# Autodesk Inventor assembly: BoronProbe_5_disassembled
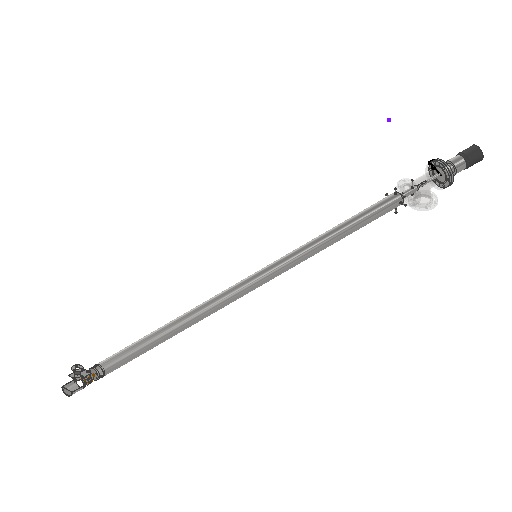
[picture p0: Inventor's stored thumbnail of the model, 512x512]
Saved by Autodesk Inventor 2026.2 (Build 302298000, 298)
## iProperties
Created: 2026-05-08
Part Number: BoronProbe_5_disassembled
Document SubType Name: Assembly
Designer: zetsu
Author: zetsu
## Documents named in this file (20)
- D:\repos\PIHTI\BoronProbe_5\BoronProbe_5_disassembled.iam
- D:\repos\PIHTI\BoronProbe_5\parts\B_probehead_5.ipt
- D:\repos\PIHTI\BoronProbe_5\parts\B_holder_sub_5.ipt
- D:\repos\PIHTI\BoronProbe_5\parts\B_pipe_cylinder_5.ipt
- D:\repos\PIHTI\BoronProbe_5\parts\B_holder_up_5.ipt
- D:\repos\PIHTI\BoronProbe_5\parts\M3-nut.ipt
- D:\repos\PIHTI\BoronProbe_5\parts\M3x6-BHCS.ipt
- D:\repos\PIHTI\BoronProbe_5\parts\substrate.ipt
- D:\repos\PIHTI\BoronProbe_5\parts\ceramic_bushing_M3-v1.ipt
- D:\repos\PIHTI\BoronProbe_5\parts\ceramic_washer_M4_v1.ipt
- D:\repos\PIHTI\BoronProbe_5\parts\B_probe_pipe_5.ipt
- D:\repos\PIHTI\BoronProbe_5\parts\B_shield_5.iam
- D:\repos\PIHTI\BoronProbe_5\parts\ceramic_2-hole-spacer_d3-13.ipt
- D:\repos\PIHTI\BoronProbe_5\parts\ceramic_spacer_d3-13.ipt
- D:\repos\PIHTI\BoronProbe_5\parts\M2-4_screw.ipt
- D:\repos\PIHTI\BoronProbe_5\parts\rotary_transfer_shaft_5.ipt
- D:\repos\PIHTI\BoronProbe_5\parts\M3x10-BHCS.ipt
- D:\repos\PIHTI\BoronProbe_5\parts\Rotary_Feedthrough\Rotary_Feedthrough.iam
- D:\repos\PIHTI\BoronProbe_5\parts\M3x20-BHCS.ipt
- D:\repos\PIHTI\BoronProbe_5\parts\ICF70TE\ICF70TE.iam
## Components (38 placed, 17 different names)
1. B_probehead_5:1 — メイト:1, メイト:2, メイト:3, メイト:4, メイト:6, メイト:12, メイト:13, メイト:14, メイト:15, メイト:16, メイト:17, メイト:18, メイト:20, メイト:22, メイト:49, メイト:50, メイト:51, メイト:52, フラッシュ:1, メイト:53, フラッシュ:2, メイト:54, フラッシュ:3
2. B_holder_sub_5:1 — メイト:1, メイト:2, メイト:3, メイト:5, メイト:7, メイト:63, メイト:64, メイト:65, メイト:66, メイト:67, メイト:68, メイト:69, メイト:70
3. Broached Hexagon Socket Button Head Cap Screw - Metric M3 x 0.5 x 6:1 — メイト:4, メイト:5
4. Broached Hexagon Socket Button Head Cap Screw - Metric M3 x 0.5 x 6:2 — メイト:6, メイト:7
5. Broached Hexagon Socket Button Head Cap Screw - Metric M3 x 0.5 x 6:5 — メイト:40, メイト:41
6. ceramic_bushing_M3-v1:1 — メイト:16, メイト:17, メイト:23, メイト:36, メイト:37
7. ceramic_bushing_M3-v1:2 — メイト:14, メイト:15, メイト:19, メイト:40, メイト:41
8. ceramic_bushing_M3-v1:3 — メイト:12, メイト:13, メイト:21, メイト:38, メイト:39
9. ceramic_washer_M4_v1:1 — メイト:20, メイト:21, メイト:43
10. ceramic_washer_M4_v1:2 — メイト:18, メイト:19, メイト:42
11. ceramic_washer_M4_v1:3 — メイト:22, メイト:23, メイト:44
12. Broached Hexagon Socket Button Head Cap Screw - Metric M3 x 0.5 x 6:6 — メイト:38, メイト:39
13. Broached Hexagon Socket Button Head Cap Screw - Metric M3 x 0.5 x 6:7 — メイト:36, メイト:37
14. B_probe_pipe_5:1 — メイト:45, メイト:46, メイト:79, メイト:80, メイト:81, メイト:82, メイト:83
15. B_pipe_cylinder_5:1 — メイト:42, メイト:43, メイト:44, メイト:45, メイト:46
16. B_shield_5:1 [sub-assembly] — メイト:49, メイト:50, メイト:51, メイト:55, メイト:56, メイト:77, メイト:78
17. ceramic_2-hole-spacer_d3-13:1 — メイト:54, フラッシュ:3
18. ceramic_spacer_d3-13:1 — メイト:53, フラッシュ:2
19. ceramic_spacer_d3-13:2 — メイト:52, フラッシュ:1
20. M2-4_screw:1 — メイト:55, メイト:77
21. M2-4_screw:2 — メイト:56, メイト:78
22. JIS B 1181 Style 1 - Metric A M3:1 — メイト:63, メイト:64
23. JIS B 1181 Style 1 - Metric A M3:2 — メイト:65, メイト:66
24. JIS B 1181 Style 1 - Metric A M3:3 — メイト:67, メイト:68
25. substrate:1 — メイト:69
26. B_holder_up_5:1 — メイト:70, メイト:71, メイト:72, メイト:73, メイト:74, メイト:75, メイト:76
27. Broached Hexagon Socket Button Head Cap Screw - Metric M3 x 0.5 x 6:8 — メイト:71, メイト:72
28. Broached Hexagon Socket Button Head Cap Screw - Metric M3 x 0.5 x 6:9 — メイト:73, メイト:74
29. Broached Hexagon Socket Button Head Cap Screw - Metric M3 x 0.5 x 6:10 — メイト:75, メイト:76
30. rotary_transfer_shaft_5:1 — メイト:79, メイト:84, 角度:1, メイト:85
31. Broached Hexagon Socket Button Head Cap Screw - Metric M3 x 0.5 x 6:11 — メイト:80
32. Broached Hexagon Socket Button Head Cap Screw - Metric M3 x 0.5 x 6:12 — メイト:81
33. Broached Hexagon Socket Button Head Cap Screw - Metric M3 x 0.5 x 6:13 — メイト:82
34. Broached Hexagon Socket Button Head Cap Screw - Metric M3 x 0.5 x 6:14 — メイト:83
35. Rotary_Feedthrough:1 [sub-assembly] — メイト:84, 角度:1, メイト:87, メイト:88, メイト:89
36. Broached Hexagon Socket Button Head Cap Screw - Metric M3 x 0.5 x 6:15 — メイト:85, メイト:86
37. JIS B 1181 Style 1 - Metric A M3:4 — メイト:86
38. ICF70TE:1 [sub-assembly] — メイト:87, メイト:88, メイト:89
## Relationships (69: Mate 65, Flush 3, Angle 1)
- メイト:1 [Mate]: B_probehead_5:1 ↔ B_holder_sub_5:1
- メイト:2 [Mate]: B_probehead_5:1 ↔ B_holder_sub_5:1
- メイト:3 [Mate]: B_probehead_5:1 ↔ B_holder_sub_5:1
- メイト:4 [Mate]: B_probehead_5:1 ↔ Broached Hexagon Socket Button Head Cap Screw - Metric M3 x 0.5 x 6:1
- メイト:5 [Mate]: B_holder_sub_5:1 ↔ Broached Hexagon Socket Button Head Cap Screw - Metric M3 x 0.5 x 6:1
- メイト:6 [Mate]: B_probehead_5:1 ↔ Broached Hexagon Socket Button Head Cap Screw - Metric M3 x 0.5 x 6:2
- メイト:7 [Mate]: B_holder_sub_5:1 ↔ Broached Hexagon Socket Button Head Cap Screw - Metric M3 x 0.5 x 6:2
- メイト:12 [Mate]: B_probehead_5:1 ↔ ceramic_bushing_M3-v1:3
- メイト:13 [Mate]: B_probehead_5:1 ↔ ceramic_bushing_M3-v1:3
- メイト:14 [Mate]: B_probehead_5:1 ↔ ceramic_bushing_M3-v1:2
- メイト:15 [Mate]: B_probehead_5:1 ↔ ceramic_bushing_M3-v1:2
- メイト:16 [Mate]: B_probehead_5:1 ↔ ceramic_bushing_M3-v1:1
- メイト:17 [Mate]: B_probehead_5:1 ↔ ceramic_bushing_M3-v1:1
- メイト:18 [Mate]: B_probehead_5:1 ↔ ceramic_washer_M4_v1:2
- メイト:19 [Mate]: ceramic_bushing_M3-v1:2 ↔ ceramic_washer_M4_v1:2
- メイト:20 [Mate]: B_probehead_5:1 ↔ ceramic_washer_M4_v1:1
- メイト:21 [Mate]: ceramic_bushing_M3-v1:3 ↔ ceramic_washer_M4_v1:1
- メイト:22 [Mate]: B_probehead_5:1 ↔ ceramic_washer_M4_v1:3
- メイト:23 [Mate]: ceramic_bushing_M3-v1:1 ↔ ceramic_washer_M4_v1:3
- メイト:36 [Mate]: ceramic_bushing_M3-v1:1 ↔ Broached Hexagon Socket Button Head Cap Screw - Metric M3 x 0.5 x 6:7
- メイト:37 [Mate]: ceramic_bushing_M3-v1:1 ↔ Broached Hexagon Socket Button Head Cap Screw - Metric M3 x 0.5 x 6:7
- メイト:38 [Mate]: ceramic_bushing_M3-v1:3 ↔ Broached Hexagon Socket Button Head Cap Screw - Metric M3 x 0.5 x 6:6
- メイト:39 [Mate]: ceramic_bushing_M3-v1:3 ↔ Broached Hexagon Socket Button Head Cap Screw - Metric M3 x 0.5 x 6:6
- メイト:40 [Mate]: Broached Hexagon Socket Button Head Cap Screw - Metric M3 x 0.5 x 6:5 ↔ ceramic_bushing_M3-v1:2
- メイト:41 [Mate]: Broached Hexagon Socket Button Head Cap Screw - Metric M3 x 0.5 x 6:5 ↔ ceramic_bushing_M3-v1:2
- メイト:42 [Mate]: ceramic_washer_M4_v1:2 ↔ B_pipe_cylinder_5:1
- メイト:43 [Mate]: ceramic_washer_M4_v1:1 ↔ B_pipe_cylinder_5:1
- メイト:44 [Mate]: ceramic_washer_M4_v1:3 ↔ B_pipe_cylinder_5:1
- メイト:45 [Mate]: B_probe_pipe_5:1 ↔ B_pipe_cylinder_5:1
- メイト:46 [Mate]: B_probe_pipe_5:1 ↔ B_pipe_cylinder_5:1
- メイト:49 [Mate]: B_probehead_5:1 ↔ B_shield_5:1
- メイト:50 [Mate]: B_probehead_5:1 ↔ B_shield_5:1
- メイト:51 [Mate]: B_probehead_5:1 ↔ B_shield_5:1
- メイト:52 [Mate]: B_probehead_5:1 ↔ ceramic_spacer_d3-13:2
- フラッシュ:1 [Flush]: B_probehead_5:1 ↔ ceramic_spacer_d3-13:2
- メイト:53 [Mate]: B_probehead_5:1 ↔ ceramic_spacer_d3-13:1
- フラッシュ:2 [Flush]: B_probehead_5:1 ↔ ceramic_spacer_d3-13:1
- メイト:54 [Mate]: B_probehead_5:1 ↔ ceramic_2-hole-spacer_d3-13:1
- フラッシュ:3 [Flush]: B_probehead_5:1 ↔ ceramic_2-hole-spacer_d3-13:1
- メイト:55 [Mate]: B_shield_5:1 ↔ M2-4_screw:1
- メイト:56 [Mate]: B_shield_5:1 ↔ M2-4_screw:2
- メイト:63 [Mate]: B_holder_sub_5:1 ↔ JIS B 1181 Style 1 - Metric A M3:1
- メイト:64 [Mate]: B_holder_sub_5:1 ↔ JIS B 1181 Style 1 - Metric A M3:1
- メイト:65 [Mate]: B_holder_sub_5:1 ↔ JIS B 1181 Style 1 - Metric A M3:2
- メイト:66 [Mate]: B_holder_sub_5:1 ↔ JIS B 1181 Style 1 - Metric A M3:2
- メイト:67 [Mate]: B_holder_sub_5:1 ↔ JIS B 1181 Style 1 - Metric A M3:3
- メイト:68 [Mate]: B_holder_sub_5:1 ↔ JIS B 1181 Style 1 - Metric A M3:3
- メイト:69 [Mate]: B_holder_sub_5:1 ↔ substrate:1
- メイト:70 [Mate]: B_holder_sub_5:1 ↔ B_holder_up_5:1
- メイト:71 [Mate]: B_holder_up_5:1 ↔ Broached Hexagon Socket Button Head Cap Screw - Metric M3 x 0.5 x 6:8
- メイト:72 [Mate]: B_holder_up_5:1 ↔ Broached Hexagon Socket Button Head Cap Screw - Metric M3 x 0.5 x 6:8
- メイト:73 [Mate]: B_holder_up_5:1 ↔ Broached Hexagon Socket Button Head Cap Screw - Metric M3 x 0.5 x 6:9
- メイト:74 [Mate]: B_holder_up_5:1 ↔ Broached Hexagon Socket Button Head Cap Screw - Metric M3 x 0.5 x 6:9
- メイト:75 [Mate]: B_holder_up_5:1 ↔ Broached Hexagon Socket Button Head Cap Screw - Metric M3 x 0.5 x 6:10
- メイト:76 [Mate]: B_holder_up_5:1 ↔ Broached Hexagon Socket Button Head Cap Screw - Metric M3 x 0.5 x 6:10
- メイト:77 [Mate]: B_shield_5:1 ↔ M2-4_screw:1
- メイト:78 [Mate]: B_shield_5:1 ↔ M2-4_screw:2
- メイト:79 [Mate]: B_probe_pipe_5:1 ↔ rotary_transfer_shaft_5:1
- メイト:80 [Mate]: B_probe_pipe_5:1 ↔ Broached Hexagon Socket Button Head Cap Screw - Metric M3 x 0.5 x 6:11
- メイト:81 [Mate]: B_probe_pipe_5:1 ↔ Broached Hexagon Socket Button Head Cap Screw - Metric M3 x 0.5 x 6:12
- メイト:82 [Mate]: B_probe_pipe_5:1 ↔ Broached Hexagon Socket Button Head Cap Screw - Metric M3 x 0.5 x 6:13
- メイト:83 [Mate]: B_probe_pipe_5:1 ↔ Broached Hexagon Socket Button Head Cap Screw - Metric M3 x 0.5 x 6:14
- メイト:84 [Mate]: rotary_transfer_shaft_5:1 ↔ Rotary_Feedthrough:1
- 角度:1 [Angle] (180 deg): rotary_transfer_shaft_5:1 ↔ Rotary_Feedthrough:1
- メイト:85 [Mate]: rotary_transfer_shaft_5:1 ↔ Broached Hexagon Socket Button Head Cap Screw - Metric M3 x 0.5 x 6:15
- メイト:86 [Mate]: Broached Hexagon Socket Button Head Cap Screw - Metric M3 x 0.5 x 6:15 ↔ JIS B 1181 Style 1 - Metric A M3:4
- メイト:87 [Mate]: Rotary_Feedthrough:1 ↔ ICF70TE:1
- メイト:88 [Mate]: Rotary_Feedthrough:1 ↔ ICF70TE:1
- メイト:89 [Mate]: Rotary_Feedthrough:1 ↔ ICF70TE:1
